# Autodesk Inventor assembly: Assembly1
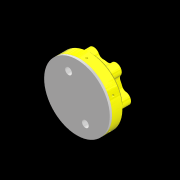
[picture p0: Inventor's stored thumbnail of the model, 180x180]
Saved by Autodesk Inventor 2020 (Build 240168000, 168)
## iProperties
Created: 2021-02-20
Part Number: Assembly1
Document SubType Name: Assembly
Designer: valer
Author: valer
## Documents named in this file (5)
- C:\Users\valer\Desktop\drummingrobot\src\parts\Encoder.iam
- C:\Users\valer\Desktop\drummingrobot\src\parts\EncoderRing.ipt
- C:\Users\valer\Desktop\drummingrobot\src\parts\EncoderBase.ipt
- C:\Users\valer\Desktop\drummingrobot\src\parts\EncoderBody.ipt
- C:\Users\valer\Desktop\drummingrobot\src\parts\external\EncoderBoard.ipt
## Components (4 placed, 4 different names)
1. EncoderRing:1 — Mate:4, Mate:5
2. EncoderBase:1 — Mate:1, Mate:2, Mate:3, Mate:6, Mate:7
3. EncoderBody:1 — Mate:4, Mate:5, Mate:6, Mate:7
4. EncoderBoard:1 — Mate:1, Mate:2, Mate:3
## Relationships (7: Mate 7)
- Mate:1: EncoderBase:1 ↔ EncoderBoard:1
- Mate:2: EncoderBase:1 ↔ EncoderBoard:1
- Mate:3: EncoderBase:1 ↔ EncoderBoard:1
- Mate:4: EncoderRing:1 ↔ EncoderBody:1
- Mate:5: EncoderRing:1 ↔ EncoderBody:1
- Mate:6: EncoderBase:1 ↔ EncoderBody:1
- Mate:7: EncoderBase:1 ↔ EncoderBody:1
